# Autodesk Inventor assembly: strikingfinal
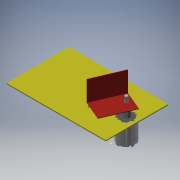
[picture p0: Inventor's stored thumbnail of the model, 180x180]
Saved by Autodesk Inventor 2019 (Build 230136000, 136)
## iProperties
Created: 2020-02-16
Part Number: strikingfinal
Document SubType Name: Assembly
Designer: Dell
Author: Dell
## Documents named in this file (4)
- C:\Users\Dell\Documents\strikingfinal.iam
- C:\Users\Dell\Documents\striking.ipt
- C:\Users\Dell\Documents\motordc2.ipt
- C:\Users\Dell\Documents\clamp3.ipt
## Components (3 placed, 3 different names)
1. striking:1 — Rotational:1
2. motordc2:1 — Rotational:1, Rigid:1
3. clamp3:1 — Rigid:1
## Relationships (2: RevoluteJoint 1, WeldJoint 1)
- Rotational:1 [RevoluteJoint]: striking:1 ↔ motordc2:1
- Rigid:1 [WeldJoint]: motordc2:1 ↔ clamp3:1
